# Autodesk Inventor assembly: Frame
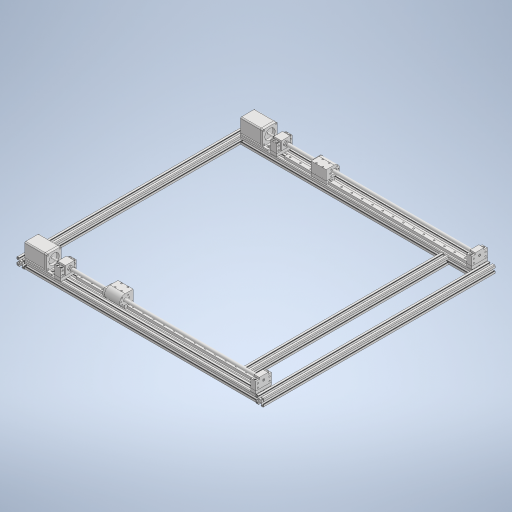
[picture p0: Inventor's stored thumbnail of the model, 512x512]
Saved by Autodesk Inventor 2023 (Build 270158000, 158)
## iProperties
Created: 2022-04-29
Part Number: Frame
Document SubType Name: Assembly
Designer: plebbb
Author: plebbb
## Documents named in this file (7)
- D:\Users\plebbb\Desktop\CNC_Project\Frame.iam
- D:\Users\plebbb\Desktop\CNC_Project\Frame_Gantry.iam
- D:\Users\plebbb\Desktop\CNC_Project\3030_Extrusion.ipt
- D:\Users\plebbb\Desktop\CNC_Project\3030_Extrusion_780.ipt
- D:\Users\plebbb\Desktop\CNC_Project\Frame_Gantry_Reverse.iam
- D:\Users\plebbb\Desktop\CNC_Project\Frame_Gantry_Carrier.iam
- D:\Users\plebbb\Desktop\CNC_Project\Frame_Gantry_Carrier_Reverse.iam
## Components (7 placed, 6 different names)
1. Frame_Gantry:1 [sub-assembly] — Mate:1, Flush:1, Flush:2, Mate:4, Flush:3, Mate:7, Flush:4
2. 3030_Extrusion:2 — Mate:1, Flush:1, Flush:2, Mate:11, Flush:10
3. 3030_Extrusion:3 — Mate:6, Flush:3, Mate:7, Flush:9, Flush:5, Mate:9
4. 3030_Extrusion_780:1 — Mate:4, Mate:6, Flush:4, Mate:10
5. Frame_Gantry_Reverse:1 [sub-assembly] — Flush:9, Flush:5, Mate:9, Mate:10, Mate:11, Flush:10
6. Frame_Gantry_Carrier:1 [sub-assembly]
7. Frame_Gantry_Carrier_Reverse:1 [sub-assembly]
## Relationships (24: Mate 13, Flush 11)
- Mate:1: Frame_Gantry:1 ↔ 3030_Extrusion:2
- Flush:1: Frame_Gantry:1 ↔ 3030_Extrusion:2
- Flush:2: Frame_Gantry:1 ↔ 3030_Extrusion:2
- Mate:4: Frame_Gantry:1 ↔ 3030_Extrusion_780:1
- Mate:6 (780 mm): 3030_Extrusion:3 ↔ 3030_Extrusion_780:1
- Flush:3: Frame_Gantry:1 ↔ 3030_Extrusion:3
- Mate:7: Frame_Gantry:1 ↔ 3030_Extrusion:3
- Flush:4: Frame_Gantry:1 ↔ 3030_Extrusion_780:1
- Flush:9: 3030_Extrusion:3 ↔ Frame_Gantry_Reverse:1
- Flush:5: 3030_Extrusion:3 ↔ Frame_Gantry_Reverse:1
- Mate:9: 3030_Extrusion:3 ↔ Frame_Gantry_Reverse:1
- Mate:10: 3030_Extrusion_780:1 ↔ Frame_Gantry_Reverse:1
- Mate:11: 3030_Extrusion:2 ↔ Frame_Gantry_Reverse:1
- Flush:10: 3030_Extrusion:2 ↔ Frame_Gantry_Reverse:1
- [Flush] (-4 mm): Frame_Gantry:1 ↔ Frame_Gantry_Carrier:1
- [Mate]: Frame_Gantry:1 ↔ Frame_Gantry_Carrier:1
- [Flush]: Frame_Gantry:1 ↔ Frame_Gantry_Carrier:1
- [Mate]: Frame_Gantry:1 ↔ Frame_Gantry_Carrier:1
- [Mate]: Frame_Gantry:1 ↔ Frame_Gantry_Carrier:1
- [Flush] (-4 mm): Frame_Gantry_Reverse:1 ↔ Frame_Gantry_Carrier_Reverse:1
- [Mate]: Frame_Gantry_Reverse:1 ↔ Frame_Gantry_Carrier_Reverse:1
- [Flush]: Frame_Gantry_Reverse:1 ↔ Frame_Gantry_Carrier_Reverse:1
- [Mate]: Frame_Gantry_Reverse:1 ↔ Frame_Gantry_Carrier_Reverse:1
- [Mate]: Frame_Gantry_Reverse:1 ↔ Frame_Gantry_Carrier_Reverse:1
## Named parameters: d13_d0 = 0 mm, d14_d2 = 0 mm, d15_d3 = 699 mm, d16_d4 = 0 mm, d3_d0 = -4 mm, d4_d1 = 0 mm, d5_d2 = 0 mm, d46_d3_d0 = -4 mm, d47_d4_d1 = 0 mm, d48_d5_d2 = 0 mm, d49_d3 = 651.2 mm, d50_d4 = 0 mm, d51_d13_d0 = 0 mm, d52_d14_d2 = 0 mm, d53_d15_d3 = 699 mm, d54_d16_d4 = 0 mm
